# Autodesk Inventor assembly: endplate_ver2111
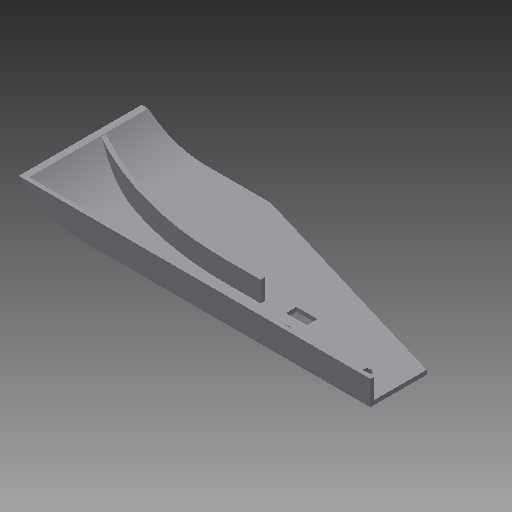
[picture p0: Inventor's stored thumbnail of the model, 512x512]
Saved by Autodesk Inventor 2018.3 (Build 223284000, 284)
## iProperties
Created: 2018-05-29
Part Number: endplate_ver2111
Material: 一般
Document SubType Name: Assembly
Designer: ku_sk
Author: ku_sk
## Documents named in this file (3)
- D:\ku_sk\ドキュメント\Inventor\Aero\KS-15\Fr.wing\parts\endplate\ver.2\endplate_ver2111.iam
- D:\ku_sk\ドキュメント\Inventor\Aero\KS-15\Fr.wing\parts\endplate\ver.2\parts\Part1111.ipt
- D:\ku_sk\ドキュメント\Inventor\Aero\KS-15\Fr.wing\parts\endplate\ver.2\parts\Part22.ipt
## Components (2 placed, 2 different names)
1. Part1111:1 — メイト:6, メイト:5, メイト:4, メイト:4, フラッシュ:1
2. Part22:1 — メイト:4, フラッシュ:1
## Relationships (5: Mate 4, Flush 1)
- メイト:6 [Mate]: Part1111:1
- メイト:5 [Mate]: Part1111:1
- メイト:4 [Mate]: Part1111:1
- メイト:4 [Mate]: Part1111:1 ↔ Part22:1
- フラッシュ:1 [Flush]: Part1111:1 ↔ Part22:1
